# Autodesk Inventor assembly: brakehandle
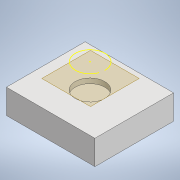
[picture p0: Inventor's stored thumbnail of the model, 180x180]
Saved by Autodesk Inventor 2021 (Build 250183000, 183)
## iProperties
Created: 2021-03-19
Part Number: brakehandle
Document SubType Name: Assembly
Designer: ben
Author: ben
## Documents named in this file (3)
- C:\Users\teh18\OneDrive\BVE Controller\r68-bve-mascon\brakehandle.iam
- C:\Users\teh18\OneDrive\BVE Controller\r68-bve-mascon\BrakeCover.ipt
- C:\Users\teh18\OneDrive\BVE Controller\r68-bve-mascon\brake\Brake-Base.ipt
## Components (2 placed, 2 different names)
1. BrakeCover:1 — Flush:1
2. Brake-Base:1 — Flush:1
## Relationships (1: Flush 1)
- Flush:1: BrakeCover:1 ↔ Brake-Base:1
